# Autodesk Inventor assembly: s-assy-link4+5+gripper
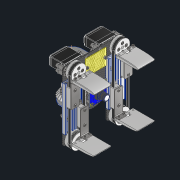
[picture p0: Inventor's stored thumbnail of the model, 180x180]
Saved by Autodesk Inventor 2021 (Build 250183000, 183)
## iProperties
Created: 2021-08-13
Part Number: s-assy-link4+5+gripper
Document SubType Name: Assembly
Designer: yuta0
Author: yuta0
## Documents named in this file (4)
- C:\Users\yuta0\Documents\GitHub\catchrobo_hardware\assy-robot\s-assy-link4+5+gripper.iam
- C:\Users\yuta0\Documents\GitHub\catchrobo_hardware\assy-robot\s-assy-gripper.iam
- C:\Users\yuta0\Documents\GitHub\catchrobo_hardware\assy-robot\s-assy-link4.iam
- C:\Users\yuta0\Documents\GitHub\catchrobo_hardware\assy-robot\base7.ipt
## Components (3 placed, 3 different names)
1. s-assy-link4:1 [sub-assembly] — メイト:1, メイト:3, メイト:4
2. s-assy-gripper:1 [sub-assembly] — メイト:2, メイト:4
3. base7:1 — メイト:1, フラッシュ:1, メイト:2, メイト:3
## Relationships (5: Mate 4, Flush 1)
- メイト:1 [Mate]: s-assy-link4:1 ↔ base7:1
- フラッシュ:1 [Flush]: base7:1
- メイト:2 [Mate]: s-assy-gripper:1 ↔ base7:1
- メイト:3 [Mate]: s-assy-link4:1 ↔ base7:1
- メイト:4 [Mate]: s-assy-link4:1 ↔ s-assy-gripper:1
